# Autodesk Inventor assembly: mount_04_mirror
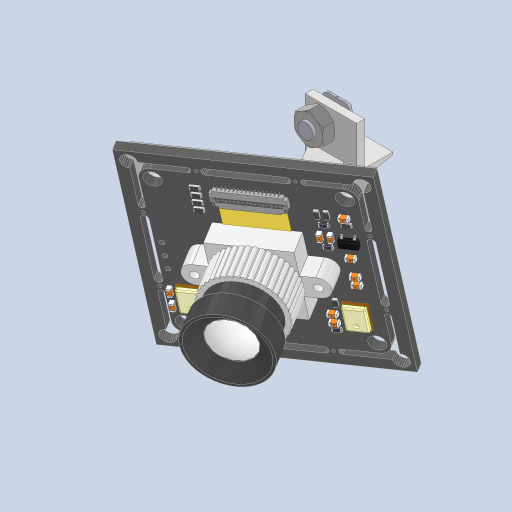
[picture p0: Inventor's stored thumbnail of the model, 512x512]
Saved by Autodesk Inventor 2024.4 (Build 284460000, 460)
## iProperties
Created: 2026-04-06
Part Number: mount_04_mirror
Document SubType Name: Assembly
Designer: tooles01
Author: tooles01
## Documents named in this file (5)
- C:\Users\tooles01\NYU Langone Health Dropbox\Shannon Toole\Shannon_Dropbox\Mar lab\RFID\camera_mount_angled\mount_04_mirror.iam
- C:\Users\tooles01\NYU Langone Health Dropbox\Shannon Toole\Shannon_Dropbox\Mar lab\Inventor_Lib\Arducam OV9281.iam
- C:\Users\tooles01\NYU Langone Health Dropbox\Shannon Toole\Shannon_Dropbox\Mar lab\Inventor_Lib\100359 M3 BO SQUARE 6.ipt
- C:\Users\tooles01\Documents\Inventor\Content Center Files\R2024\en-US\AS 1112 (2)\AS 1112 - M3  Type 5.ipt
- C:\Users\tooles01\NYU Langone Health Dropbox\Shannon Toole\Shannon_Dropbox\Mar lab\RFID\camera_mount_angled\angle_04_mirror.ipt
## Components (4 placed, 4 different names)
1. Arducam OV9281:1 [sub-assembly] — cam screw:1, cam screw:2
2. angle_04_mirror:1 — cam screw:1, cam screw:2, M3 to angle piece, nut flush to angle piece
3. 100359 M3 BO SQUARE 6:1 — M3 to angle piece, nut to screw
4. AS 1112 (2) - Metric M3  Type 5:1 — nut flush to angle piece, nut to screw
## Relationships (5: Mate 3, Insert 2)
- cam screw:1 [Insert]: Arducam OV9281:1 ↔ angle_04_mirror:1
- cam screw:2 [Insert]: Arducam OV9281:1 ↔ angle_04_mirror:1
- M3 to angle piece [Mate]: angle_04_mirror:1 ↔ 100359 M3 BO SQUARE 6:1
- nut flush to angle piece [Mate]: angle_04_mirror:1 ↔ AS 1112 (2) - Metric M3  Type 5:1
- nut to screw [Mate]: 100359 M3 BO SQUARE 6:1 ↔ AS 1112 (2) - Metric M3  Type 5:1
